# Autodesk Inventor assembly: robot_top
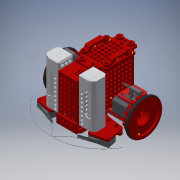
[picture p0: Inventor's stored thumbnail of the model, 180x180]
Saved by Autodesk Inventor 2016 (Build 200138000, 138)
## iProperties
Created: 2016-02-13
Part Number: robot_top
Document SubType Name: Assembly
Designer: jforce
Author: jforce
## Documents named in this file (12)
- C:\Users\jforce\Dropbox\gmu\ece590\maze-robot\robot_top.iam
- C:\Users\jforce\Dropbox\gmu\ece590\maze-robot\chassis_plate.ipt
- C:\Users\jforce\Dropbox\gmu\ece590\maze-robot\robotis_pi_box.iam
- C:\Users\jforce\Dropbox\gmu\ece590\maze-robot\r_wheel_assembly.iam
- C:\Users\jforce\Dropbox\gmu\ece590\maze-robot\l_wheel_assembly.iam
- C:\Users\jforce\Dropbox\gmu\ece590\maze-robot\opencm9_grp.iam
- C:\Users\jforce\Dropbox\gmu\ece590\maze-robot\batt.iam
- C:\Users\jforce\Dropbox\gmu\ece590\maze-robot\batt_MIR1.iam
- C:\Users\jforce\Dropbox\gmu\ece590\maze-robot\bumper.iam
- C:\Users\jforce\Dropbox\gmu\ece590\maze-robot\caster_pad.ipt
- C:\Users\jforce\Dropbox\gmu\ece590\maze-robot\bumper_wire.ipt
- C:\Users\jforce\Dropbox\gmu\ece590\maze-robot\bumper_wire_MIR.ipt
## Components (11 placed, 11 different names)
1. chassis_plate:1 — Mate:23, Mate:26, Mate:27, Mate:28, Mate:29, Mate:30, Mate:32
2. robotis_pi_box:1 [sub-assembly] — Mate:29, Mate:31, Mate:32, Mate:34, Mate:35, Mate:36, Mate:37, Mate:38, Angle:1, Symmetry:1
3. r_wheel_assembly:1 [sub-assembly] — Mate:26, Mate:27, Mate:28
4. l_wheel_assembly:1 [sub-assembly] — Mate:23, Mate:30, Mate:44
5. opencm9_grp:1 [sub-assembly] — Mate:31, Mate:37
6. batt:2 [sub-assembly] — Mate:34, Mate:35, Mate:36
7. batt_MIR1:1 [sub-assembly]
8. bumper:1 [sub-assembly] — Mate:40, Mate:41, Mate:42, Mate:43, Mate:48
9. caster_pad:1 — Mate:40, Mate:41, Mate:42, Mate:43
10. bumper_wire:1
11. bumper_wire_MIR:1
## Relationships (26: Mate 23, Angle 2, Symmetry 1)
- Mate:23: chassis_plate:1 ↔ l_wheel_assembly:1
- Mate:26: chassis_plate:1 ↔ r_wheel_assembly:1
- Mate:27: chassis_plate:1 ↔ r_wheel_assembly:1
- Mate:28: chassis_plate:1 ↔ r_wheel_assembly:1
- Mate:29: chassis_plate:1 ↔ robotis_pi_box:1
- Mate:30: chassis_plate:1 ↔ l_wheel_assembly:1
- Mate:31: robotis_pi_box:1 ↔ opencm9_grp:1
- Mate:32: chassis_plate:1 ↔ robotis_pi_box:1
- Mate:34: robotis_pi_box:1 ↔ batt:2
- Mate:35: robotis_pi_box:1 ↔ batt:2
- Mate:36: robotis_pi_box:1 ↔ batt:2
- Mate:37: robotis_pi_box:1 ↔ opencm9_grp:1
- Mate:38: robotis_pi_box:1
- Angle:1 (0 deg): robotis_pi_box:1
- Symmetry:1: robotis_pi_box:1
- Mate:40: bumper:1 ↔ caster_pad:1
- Mate:41: bumper:1 ↔ caster_pad:1
- Mate:42: bumper:1 ↔ caster_pad:1
- Mate:43: bumper:1 ↔ caster_pad:1
- Mate:44: l_wheel_assembly:1
- Mate:45
- Mate:46
- Mate:47
- Angle:3 (0 deg)
- Mate:48: bumper:1
- Mate:49
